# Autodesk Inventor assembly: motor-and-drive
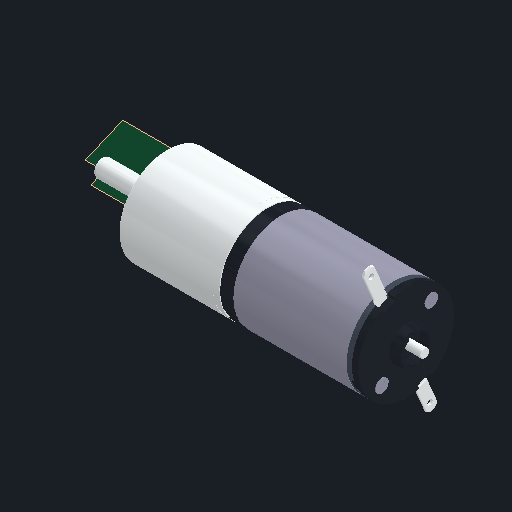
[picture p0: Inventor's stored thumbnail of the model, 512x512]
Saved by Autodesk Inventor 2026.1 (Build 301233020, 233B)
## iProperties
Company: CADClick - www.CADClick.com
Created: 2026-02-25
Part Number: motor-and-drive
Description: STEP AP214
Document SubType Name: Assembly
Designer: Jan
Authority: unknown authorization
Preprocessor: Spatial InterOp 3D
Title: cctmp_49F80096-2CC1-42B4-8485-2F1183888B6A_2026_2_25_18_2_20_911..stp
Author: maxon motor ag
Revision Number: NONE
## Documents named in this file (11)
- C:\Users\Jan\OneDrive\Pulpit\Ainventor-ZNL\czesci\motor-and-drive\motor-and-drive\motor-and-drive.iam
- C:\Users\Jan\OneDrive\Pulpit\Ainventor-ZNL\czesci\motor-and-drive\motor-and-drive\0.ipt
- C:\Users\Jan\OneDrive\Pulpit\Ainventor-ZNL\czesci\motor-and-drive\motor-and-drive\0_1.ipt
- C:\Users\Jan\OneDrive\Pulpit\Ainventor-ZNL\czesci\motor-and-drive\motor-and-drive\0_2.ipt
- C:\Users\Jan\OneDrive\Pulpit\Ainventor-ZNL\czesci\motor-and-drive\motor-and-drive\0_3.ipt
- C:\Users\Jan\OneDrive\Pulpit\Ainventor-ZNL\czesci\motor-and-drive\motor-and-drive\0_4.ipt
- C:\Users\Jan\OneDrive\Pulpit\Ainventor-ZNL\czesci\motor-and-drive\motor-and-drive\0_5.ipt
- C:\Users\Jan\OneDrive\Pulpit\Ainventor-ZNL\czesci\motor-and-drive\motor-and-drive\0_6.ipt
- C:\Users\Jan\OneDrive\Pulpit\Ainventor-ZNL\czesci\motor-and-drive\motor-and-drive\0_7.ipt
- C:\Users\Jan\OneDrive\Pulpit\Ainventor-ZNL\czesci\motor-and-drive\motor-and-drive\0_8.ipt
- C:\Users\Jan\OneDrive\Pulpit\Ainventor-ZNL\czesci\motor-and-drive\motor-and-drive\0_9.ipt
## Components (10 placed, 10 different names)
1. 0 — Angle:1, Tangent:1, Mate:1, Mate:5
2. 0_1
3. 0_2 — Mate:1, Mate:2, Mate:4
4. 0_3 — Mate:2
5. 0_4
6. 0_5
7. 0_6
8. 0_7
9. 0_8
10. 0_9
## Relationships (9: Mate 6, Angle 2, Tangent 1)
- Angle:1 (0 deg): 0
- Tangent:1: 0
- Mate:1: 0 ↔ 0_2
- Mate:2: 0_2 ↔ 0_3
- Mate:4: 0_2
- Mate:5: 0
- Mate:6
- Mate:7
- Angle:2 (0 deg)
